# Autodesk Inventor assembly: FrameInternals
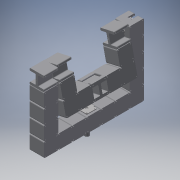
[picture p0: Inventor's stored thumbnail of the model, 180x180]
Saved by Autodesk Inventor 2016 (Build 200138000, 138)
## iProperties
Created: 2016-05-22
Part Number: FrameInternals
Document SubType Name: Assembly
Designer: Kurtis
Author: Kurtis
## Documents named in this file (3)
- C:\Users\Kurtis\Git\CAD\Sentry Camera\cad\FrameInternals.iam
- C:\Users\Kurtis\Git\CAD\Sentry Camera\cad\OuterFrameInternals.iam
- C:\Users\Kurtis\Git\CAD\Sentry Camera\cad\InnerFrameInternals.iam
## Components (2 placed, 2 different names)
1. OuterFrameInternals:1 [sub-assembly] — Cylindrical:1
2. InnerFrameInternals:1 [sub-assembly] — Cylindrical:1
## Relationships (1: CylindricalJoint 1)
- Cylindrical:1: OuterFrameInternals:1 ↔ InnerFrameInternals:1
